# Autodesk Inventor assembly: Carriage_Assembly
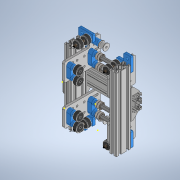
[picture p0: Inventor's stored thumbnail of the model, 180x180]
Saved by Autodesk Inventor 2021 (Build 250183000, 183)
## iProperties
Created: 2021-09-08
Part Number: Carriage_Assembly
Document SubType Name: Assembly
Designer: Jorian Brusind
Author: Jorian Brusind
## Documents named in this file (11)
- C:\Users\Jorian Bruslind\Documents\GitHub\PersonalProjects\HyperRail\Inventor Files\Carriage_Assembly.iam
- C:\Users\Jorian Bruslind\Documents\GitHub\PersonalProjects\Inventor Projects\Useful models\8020_Sets\IPT_20_Series\IPT_20_Series\20-2040_200mm.ipt
- C:\Users\Jorian Bruslind\Documents\GitHub\PersonalProjects\Inventor Projects\Useful models\8020_Sets\IPT_20_Series\IPT_20_Series\20-2040_150mm.ipt
- C:\Users\Jorian Bruslind\Documents\GitHub\PersonalProjects\HyperRail\Inventor Files\X_CarriageL_V2_0_Short.iam
- C:\Users\Jorian Bruslind\Documents\GitHub\PersonalProjects\HyperRail\Inventor Files\X_CarriageR_V2_0_Short.iam
- C:\Users\Jorian Bruslind\Documents\GitHub\PersonalProjects\HyperRail\Inventor Files\X_CarriageR_V2_0.iam
- C:\Users\Jorian Bruslind\Documents\GitHub\PersonalProjects\HyperRail\Inventor Files\X_Carriage_V2_0.iam
- C:\Users\Jorian Bruslind\Documents\GitHub\PersonalProjects\Inventor Projects\Useful models\8020_Sets\IPT_20_Series\Extra_20_Series\8020_14056m\14056_m.ipt
- C:\Users\Jorian Bruslind\Documents\GitHub\PersonalProjects\HyperRail\Inventor Files\Buffer.iam
- C:\Users\Jorian Bruslind\Documents\GitHub\PersonalProjects\Inventor Projects\Useful models\Metric Spacer_Standoffs\hex spacer standoff nut M5 L30.ipt
- C:\Users\Jorian Bruslind\Documents\GitHub\PersonalProjects\HyperRail\Inventor Files\Carriage_Horizontal_Spacer.ipt
## Components (23 placed, 10 different names)
1. 20-2040_200mm:1 — Mate:1, Flush:1, Mate:2, Flush:2, Mate:3, Mate:4, Mate:5, Mate:6, Mate:7, Flush:3, Mate:9, Flush:6, Flush:7, Flush:11, Flush:12, Mate:51, Flush:18, Mate:53, Flush:22, Flush:24, Mate:69
2. 20-2040_200mm:2 — Mate:10, Mate:11, Flush:5, Flush:6, Flush:7, Flush:9, Flush:10, Mate:52, Flush:20, Flush:21, Mate:56, Flush:23, Flush:28, Mate:71, Flush:29, Flush:30
3. 20-2040_150mm:1 — Flush:3, Mate:8, Mate:9, Mate:20, Mate:21, Mate:22, Mate:23
4. X_CarriageL_V2_0_Short:1 [sub-assembly] — Mate:10, Flush:5, Mate:57, Mate:65, Mate:68, Flush:29
5. X_CarriageR_V2_0_Short:1 [sub-assembly] — Mate:11, Mate:59, Mate:60, Mate:63, Flush:30
6. X_CarriageR_V2_0:1 [sub-assembly] — Mate:1, Flush:1, Mate:2, Mate:8, Mate:54, Mate:64, Mate:66, Mate:67
7. X_Carriage_V2_0:1 [sub-assembly] — Flush:2, Mate:3, Mate:4, Mate:55, Mate:58, Mate:61, Mate:62
8. 14056_m:1 — Mate:21, Flush:9, Mate:72
9. 14056_m:2 — Mate:20, Flush:10, Flush:27, Mate:73
10. 14056_m:3 — Mate:22, Flush:12, Flush:25, Flush:26
11. 14056_m:4 — Mate:23, Flush:11, Flush:26, Mate:70
12. Buffer:1 [sub-assembly] — Mate:56, Flush:23, Mate:57
13. Buffer:2 [sub-assembly] — Mate:53, Flush:22, Mate:54
14. Buffer:3 [sub-assembly] — Mate:52, Flush:20, Flush:21
15. Buffer:4 [sub-assembly] — Mate:51, Flush:18, Mate:55
16. hex spacer standoff nut M5 L30:1
17. hex spacer standoff nut M5 L30:2 — Mate:64, Mate:65, Mate:66
18. hex spacer standoff nut M5 L30:3 — Mate:67, Mate:68
19. hex spacer standoff nut M5 L30:4 — Mate:62, Mate:63
20. hex spacer standoff nut M5 L30:5
21. hex spacer standoff nut M5 L30:6 — Mate:58, Mate:59, Mate:60, Mate:61
22. Carriage_Horizontal_Spacer:1 — Flush:24, Mate:69, Flush:25, Mate:70
23. Carriage_Horizontal_Spacer:2 — Flush:27, Flush:28, Mate:71, Mate:72, Mate:73
## Relationships (60: Mate 38, Flush 22)
- Mate:1: 20-2040_200mm:1 ↔ X_CarriageR_V2_0:1
- Flush:1: 20-2040_200mm:1 ↔ X_CarriageR_V2_0:1
- Mate:2 (5 mm): 20-2040_200mm:1 ↔ X_CarriageR_V2_0:1
- Flush:2: 20-2040_200mm:1 ↔ X_Carriage_V2_0:1
- Mate:3: 20-2040_200mm:1 ↔ X_Carriage_V2_0:1
- Mate:4 (5 mm): 20-2040_200mm:1 ↔ X_Carriage_V2_0:1
- Mate:5: 20-2040_200mm:1
- Mate:6: 20-2040_200mm:1
- Mate:7: 20-2040_200mm:1
- Flush:3: 20-2040_200mm:1 ↔ 20-2040_150mm:1
- Mate:8 (5 mm): 20-2040_150mm:1 ↔ X_CarriageR_V2_0:1
- Mate:9 (5 mm): 20-2040_200mm:1 ↔ 20-2040_150mm:1
- Mate:10: 20-2040_200mm:2 ↔ X_CarriageL_V2_0_Short:1
- Mate:11: 20-2040_200mm:2 ↔ X_CarriageR_V2_0_Short:1
- Flush:5: 20-2040_200mm:2 ↔ X_CarriageL_V2_0_Short:1
- Flush:6: 20-2040_200mm:1 ↔ 20-2040_200mm:2
- Flush:7: 20-2040_200mm:1 ↔ 20-2040_200mm:2
- Mate:20: 20-2040_150mm:1 ↔ 14056_m:2
- Mate:21: 20-2040_150mm:1 ↔ 14056_m:1
- Flush:9: 20-2040_200mm:2 ↔ 14056_m:1
- Flush:10: 20-2040_200mm:2 ↔ 14056_m:2
- Mate:22: 20-2040_150mm:1 ↔ 14056_m:3
- Mate:23: 20-2040_150mm:1 ↔ 14056_m:4
- Flush:11: 20-2040_200mm:1 ↔ 14056_m:4
- Flush:12: 20-2040_200mm:1 ↔ 14056_m:3
- Mate:51: 20-2040_200mm:1 ↔ Buffer:4
- Flush:18: 20-2040_200mm:1 ↔ Buffer:4
- Mate:52: 20-2040_200mm:2 ↔ Buffer:3
- Flush:20: 20-2040_200mm:2 ↔ Buffer:3
- Flush:21: 20-2040_200mm:2 ↔ Buffer:3
- Mate:53: 20-2040_200mm:1 ↔ Buffer:2
- Flush:22: 20-2040_200mm:1 ↔ Buffer:2
- Mate:54: X_CarriageR_V2_0:1 ↔ Buffer:2
- Mate:55: X_Carriage_V2_0:1 ↔ Buffer:4
- Mate:56: 20-2040_200mm:2 ↔ Buffer:1
- Flush:23: 20-2040_200mm:2 ↔ Buffer:1
- Mate:57: X_CarriageL_V2_0_Short:1 ↔ Buffer:1
- Mate:58: X_Carriage_V2_0:1 ↔ hex spacer standoff nut M5 L30:6
- Mate:59: X_CarriageR_V2_0_Short:1 ↔ hex spacer standoff nut M5 L30:6
- Mate:60: X_CarriageR_V2_0_Short:1 ↔ hex spacer standoff nut M5 L30:6
- Mate:61: X_Carriage_V2_0:1 ↔ hex spacer standoff nut M5 L30:6
- Mate:62: X_Carriage_V2_0:1 ↔ hex spacer standoff nut M5 L30:4
- Mate:63: X_CarriageR_V2_0_Short:1 ↔ hex spacer standoff nut M5 L30:4
- Mate:64: X_CarriageR_V2_0:1 ↔ hex spacer standoff nut M5 L30:2
- Mate:65: X_CarriageL_V2_0_Short:1 ↔ hex spacer standoff nut M5 L30:2
- Mate:66: X_CarriageR_V2_0:1 ↔ hex spacer standoff nut M5 L30:2
- Mate:67: X_CarriageR_V2_0:1 ↔ hex spacer standoff nut M5 L30:3
- Mate:68: X_CarriageL_V2_0_Short:1 ↔ hex spacer standoff nut M5 L30:3
- Flush:24: 20-2040_200mm:1 ↔ Carriage_Horizontal_Spacer:1
- Mate:69: 20-2040_200mm:1 ↔ Carriage_Horizontal_Spacer:1
- Flush:25: 14056_m:3 ↔ Carriage_Horizontal_Spacer:1
- Flush:26: 14056_m:3 ↔ 14056_m:4
- Mate:70: 14056_m:4 ↔ Carriage_Horizontal_Spacer:1
- Flush:27: 14056_m:2 ↔ Carriage_Horizontal_Spacer:2
- Flush:28: 20-2040_200mm:2 ↔ Carriage_Horizontal_Spacer:2
- Mate:71: 20-2040_200mm:2 ↔ Carriage_Horizontal_Spacer:2
- Mate:72: 14056_m:1 ↔ Carriage_Horizontal_Spacer:2
- Mate:73: 14056_m:2 ↔ Carriage_Horizontal_Spacer:2
- Flush:29: 20-2040_200mm:2 ↔ X_CarriageL_V2_0_Short:1
- Flush:30: 20-2040_200mm:2 ↔ X_CarriageR_V2_0_Short:1
